# Autodesk Inventor assembly: ASY Beshkino_bio_tank
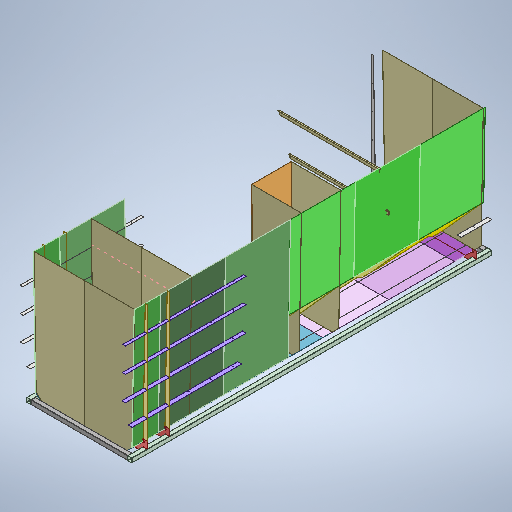
[picture p0: Inventor's stored thumbnail of the model, 512x512]
Saved by Autodesk Inventor 2025 (Build 290162010, 162A)
## iProperties
Created: 2024-07-21
Part Number: ASY Beshkino_bio_tank
Document SubType Name: Assembly
Designer: admin
Mass: 5.81287e+06 g
Surface Area: 2.77755e+06 cm^2
Volume: 3.12018e+06 cm^3
Density: 1.86299 g/cm^3
Author: admin
## Documents named in this file (29)
- C:\Users\user\YandexDisk\домашниий пк\Inventor\BSH_Beshkino_bio_tank\ASY Beshkino_bio_tank.iam
- C:\Users\user\YandexDisk\домашниий пк\Inventor\BSH_Beshkino_bio_tank\BSH 000 dim Beshkino_bio_tank.ipt
- C:\Users\user\YandexDisk\домашниий пк\Inventor\BSH_Beshkino_bio_tank\BSH 010 floor 1.ipt
- C:\Users\user\YandexDisk\домашниий пк\Inventor\BSH_Beshkino_bio_tank\BSH 021 rib 1.ipt
- C:\Users\user\YandexDisk\домашниий пк\Inventor\BSH_Beshkino_bio_tank\BSH 022 rib 2.ipt
- C:\Users\user\YandexDisk\домашниий пк\Inventor\BSH_Beshkino_bio_tank\BSH 061 tube 1.ipt
- C:\Users\user\YandexDisk\домашниий пк\Inventor\BSH_Beshkino_bio_tank\BSH 031 nose 1.ipt
- C:\Users\user\YandexDisk\домашниий пк\Inventor\BSH_Beshkino_bio_tank\BSH 032 board 2.ipt
- C:\Users\user\YandexDisk\домашниий пк\Inventor\BSH_Beshkino_bio_tank\BSH 033 board 3.ipt
- C:\Users\user\YandexDisk\домашниий пк\Inventor\BSH_Beshkino_bio_tank\BSH 041 stringer 1.ipt
- C:\Users\user\YandexDisk\домашниий пк\Inventor\BSH_Beshkino_bio_tank\BSH 039 back 9.ipt
- C:\Users\user\YandexDisk\домашниий пк\Inventor\BSH_Beshkino_bio_tank\BSH 041 stringer floor.ipt
- C:\Users\user\YandexDisk\домашниий пк\Inventor\BSH_Beshkino_bio_tank\BSH 062 tube 2.ipt
- C:\Users\user\YandexDisk\домашниий пк\Inventor\BSH_Beshkino_bio_tank\BSH 042 stringer 2.ipt
- C:\Users\user\YandexDisk\домашниий пк\Inventor\BSH_Beshkino_bio_tank\BSH 043 stringer 3.ipt
- C:\Users\user\YandexDisk\домашниий пк\Inventor\BSH_Beshkino_bio_tank\BSH 044 stringer 4.ipt
- C:\Users\user\YandexDisk\домашниий пк\Inventor\BSH_Beshkino_bio_tank\BSH 020 rib 1.ipt
- C:\Users\user\YandexDisk\домашниий пк\Inventor\BSH_Beshkino_bio_tank\BSH 042 stringer floor.ipt
- C:\Users\user\YandexDisk\домашниий пк\Inventor\BSH_Beshkino_bio_tank\BSH 045 stringer 1.ipt
- C:\Users\user\YandexDisk\домашниий пк\Inventor\BSH_Beshkino_bio_tank\BSH 045 stringer 5.ipt
- C:\Users\user\YandexDisk\домашниий пк\Inventor\BSH_Beshkino_bio_tank\BSH 033 board cone 3.ipt
- C:\Users\user\YandexDisk\домашниий пк\Inventor\BSH_Beshkino_bio_tank\BSH 034 board cone 4.ipt
- C:\Users\user\YandexDisk\домашниий пк\Inventor\BSH_Beshkino_bio_tank\BSH 035 divider 1.ipt
- C:\Users\user\YandexDisk\домашниий пк\Inventor\BSH_Beshkino_bio_tank\BSH 036 divider 2.ipt
- C:\Users\user\YandexDisk\домашниий пк\Inventor\BSH_Beshkino_bio_tank\BSH 012 floor 2.ipt
- C:\Users\user\YandexDisk\домашниий пк\Inventor\BSH_Beshkino_bio_tank\BSH 037 cone 3.ipt
- C:\Users\user\YandexDisk\домашниий пк\Inventor\BSH_Beshkino_bio_tank\BSH 013 floor 3.ipt
- C:\Users\user\YandexDisk\домашниий пк\Inventor\BSH_Beshkino_bio_tank\BSH 015 board cone 5.ipt
- C:\Users\user\YandexDisk\домашниий пк\Inventor\BSH_Beshkino_bio_tank\BSH 038 divider.ipt
## Components (70 placed, 34 different names)
1. BSH 000 dim Beshkino_bio_tank.ipt:1
2. BSH 022 rib 2.ipt:1 — Rigid:3, Mate:8, Rigid:27, Rigid:28, Rigid:29, Rigid:30
3. BSH 061 tube 1.ipt:1 — Mate:1, Rigid:1, Mate:3
4. BSH 061 tube 1.ipt:2 — Mate:2, Rigid:1, Mate:4, Flush:3, Flush:4, Rigid:14, Rigid:15, Mate:20, Mate:21
5. BSH 062 tube 2.ipt:1 — Rigid:14, Mate:19
6. BSH 062 tube 2.ipt:2 — Rigid:15
7. BSH 010 floor 1.ipt:2 — Rigid:4, Rigid:5, Mate:39
8. BSH 010 floor 1.ipt:3 — Rigid:5, Mate:9, Rigid:65, Mate:47, Mate:54
9. BSH 010 floor 1.ipt:1 — Mate:5, Mate:6, Rigid:4, Mate:7, Flush:4, Mate:10, Flush:5, Flush:11
10. BSH 031 nose 1.ipt:1 — Mate:10, Flush:5, Mate:11, Rigid:11
11. BSH 032 board 2.ipt:1 — Mate:8, Mate:9, Rigid:8, Rigid:58
12. BSH 033 board 3.ipt:1 — Rigid:8, Flush:10, Flush:11
13. BSH 031 nose 1.ipt:2 — Rigid:11, Rigid:53
14. BSH 039 back 9.ipt:1 — Rigid:68, Rigid:69
15. BSH 022 rib 2.ipt:2 — Rigid:16, Rigid:31, Rigid:32, Rigid:33, Rigid:34, Mate:38
16. BSH 021 rib 1.ipt:1 — Mate:4, Flush:3, Mate:5, Mate:6, Rigid:3, Rigid:9, Rigid:16, Rigid:20, Rigid:22, Rigid:24, Rigid:26, Mate:19
17. BSH 041 stringer floor.ipt:2 — Rigid:22, Rigid:41
18. BSH 041 stringer floor.ipt:3 — Rigid:24, Rigid:42
19. BSH 041 stringer floor.ipt:4 — Rigid:26, Rigid:43
20. BSH 041 stringer floor.ipt:5 — Rigid:35, Rigid:36
21. BSH 041 stringer floor.ipt:6 — Rigid:36
22. BSH 041 stringer floor:10 — Rigid:41
23. BSH 041 stringer floor:11
24. BSH 041 stringer floor:12 — Rigid:42
25. BSH 041 stringer floor:14 — Rigid:43
26. BSH 041 stringer floor:13
27. BSH 041 stringer floor:15
28. BSH 041 stringer floor.ipt:1 — Rigid:20, Rigid:35
29. BSH 042 stringer floor:1 — Rigid:37
30. BSH 042 stringer floor:2 — Rigid:44
31. BSH 042 stringer floor:3 — Rigid:45
32. BSH 042 stringer floor:4 — Rigid:46
33. BSH 020 rib 1:4 — Mate:20, Mate:21, Rigid:37, Rigid:44, Rigid:45, Rigid:46, Rigid:48
34. BSH 022 rib 2:32 — Rigid:48
35. BSH 045 stringer 1:1
36. BSH 045 stringer 5:1 — Mate:22, Mate:23
37. BSH 031 nose 1:3 — Rigid:55, Mate:22
38. BSH 031 nose 1:4 — Rigid:53
39. BSH 031 nose 1:5 — Rigid:54, Mate:29, Mate:41, Mate:48, Mate:51, Mate:56, Mate:57
40. BSH 031 nose 1:6 — Rigid:54, Rigid:55, Mate:55
41. BSH 033 board cone 3:1 — Mate:26, Rigid:57, Mate:30
42. BSH 031 nose 1:7 — Mate:26, Mate:30
43. BSH 031 nose 1:8 — Flush:8, Mate:40
44. BSH 033 board cone 3:2 — Rigid:57, Mate:29, Mate:41, Mate:46, Angle:1, Mate:49, Mate:50, Mate:52
45. BSH 032 board 2:2 — Rigid:58, Rigid:68
46. BSH 022 rib 2.ipt:3 — Rigid:17
47. BSH 021 rib 1.ipt:2 — Rigid:9, Rigid:17, Rigid:18
48. BSH 022 rib 2.ipt:4 — Rigid:18
49. BSH 044 stringer 4.ipt:1 — Rigid:30
50. BSH 043 stringer 3.ipt:1 — Rigid:29
51. BSH 042 stringer 2.ipt:1 — Rigid:28
52. BSH 041 stringer 1.ipt:1 — Rigid:27
53. BSH 041 stringer 1.ipt:2 — Rigid:31
54. BSH 042 stringer 2.ipt:2 — Rigid:32
55. BSH 043 stringer 3.ipt:2 — Rigid:33
56. BSH 044 stringer 4.ipt:2 — Rigid:34
57. BSH 034 board cone 4:1 — Rigid:62, Mate:43, Mate:51, Mate:52, Mate:53
58. BSH 034 board cone 4:2 — Rigid:62
59. BSH 035 divider 1:1 — Mate:44
60. BSH 036 divider 2:1
61. BSH 012 floor 2:1 — Rigid:65, Rigid:66, Mate:42, Angle:1, Mate:49, Mate:53
62. BSH 037 cone 3:1 — Mate:42, Mate:43, Mate:50
63. BSH 033 board 3:2 — Rigid:64, Flush:10
64. BSH 012 floor 2:2 — Rigid:66, Rigid:67
65. BSH 013 floor 3:1 — Rigid:67, Mate:40
66. BSH 039 back 9:2 — Rigid:69, Rigid:70
67. BSH 039 back 9:3 — Rigid:70
68. BSH 015 board cone 5:1 — Mate:46, Mate:47, Mate:48
69. BSH 038 divider:1 — Mate:54, Mate:55, Mate:56, Mate:57
70. BSH 032 board 2:4 — Mate:38, Mate:39, Rigid:64
## Component patterns: (1 elements, first: BSH 032 board 2:4)
## Relationships (97: WeldJoint 52, Mate 38, Flush 6, Angle 1)
- Mate:1: BSH 061 tube 1.ipt:1
- Mate:2: BSH 061 tube 1.ipt:2
- Rigid:1 [WeldJoint] (-2400 mm): BSH 061 tube 1.ipt:1 ↔ BSH 061 tube 1.ipt:2
- Mate:3: BSH 061 tube 1.ipt:1
- Mate:4: BSH 061 tube 1.ipt:2 ↔ BSH 021 rib 1.ipt:1
- Flush:3: BSH 061 tube 1.ipt:2 ↔ BSH 021 rib 1.ipt:1
- Mate:5: BSH 010 floor 1.ipt:1 ↔ BSH 021 rib 1.ipt:1
- Mate:6: BSH 010 floor 1.ipt:1 ↔ BSH 021 rib 1.ipt:1
- Rigid:3 [WeldJoint]: BSH 022 rib 2.ipt:1 ↔ BSH 021 rib 1.ipt:1
- Rigid:4 [WeldJoint]: BSH 010 floor 1.ipt:2 ↔ BSH 010 floor 1.ipt:1
- Rigid:5 [WeldJoint]: BSH 010 floor 1.ipt:2 ↔ BSH 010 floor 1.ipt:3
- Mate:7: BSH 010 floor 1.ipt:1
- Flush:4 (100 mm): BSH 061 tube 1.ipt:2 ↔ BSH 010 floor 1.ipt:1
- Mate:8: BSH 022 rib 2.ipt:1 ↔ BSH 032 board 2.ipt:1
- Mate:9: BSH 010 floor 1.ipt:3 ↔ BSH 032 board 2.ipt:1
- Rigid:8 [WeldJoint]: BSH 032 board 2.ipt:1 ↔ BSH 033 board 3.ipt:1
- Rigid:9 [WeldJoint] (-500 mm): BSH 021 rib 1.ipt:1 ↔ BSH 021 rib 1.ipt:2
- Mate:10: BSH 010 floor 1.ipt:1 ↔ BSH 031 nose 1.ipt:1
- Flush:5 (10 mm): BSH 010 floor 1.ipt:1 ↔ BSH 031 nose 1.ipt:1
- Mate:11: BSH 031 nose 1.ipt:1
- Rigid:11 [WeldJoint]: BSH 031 nose 1.ipt:1 ↔ BSH 031 nose 1.ipt:2
- Rigid:14 [WeldJoint]: BSH 061 tube 1.ipt:2 ↔ BSH 062 tube 2.ipt:1
- Rigid:15 [WeldJoint]: BSH 061 tube 1.ipt:2 ↔ BSH 062 tube 2.ipt:2
- Rigid:16 [WeldJoint]: BSH 022 rib 2.ipt:2 ↔ BSH 021 rib 1.ipt:1
- Rigid:17 [WeldJoint]: BSH 022 rib 2.ipt:3 ↔ BSH 021 rib 1.ipt:2
- Rigid:18 [WeldJoint]: BSH 021 rib 1.ipt:2 ↔ BSH 022 rib 2.ipt:4
- Rigid:20 [WeldJoint] (2 mm): BSH 021 rib 1.ipt:1 ↔ BSH 041 stringer floor.ipt:1
- Rigid:22 [WeldJoint] (2 mm): BSH 021 rib 1.ipt:1 ↔ BSH 041 stringer floor.ipt:2
- Rigid:24 [WeldJoint]: BSH 021 rib 1.ipt:1 ↔ BSH 041 stringer floor.ipt:3
- Rigid:26 [WeldJoint] (2 mm): BSH 021 rib 1.ipt:1 ↔ BSH 041 stringer floor.ipt:4
- Rigid:27 [WeldJoint] (2 mm): BSH 022 rib 2.ipt:1 ↔ BSH 041 stringer 1.ipt:1
- Rigid:28 [WeldJoint] (2 mm): BSH 022 rib 2.ipt:1 ↔ BSH 042 stringer 2.ipt:1
- Rigid:29 [WeldJoint] (2 mm): BSH 022 rib 2.ipt:1 ↔ BSH 043 stringer 3.ipt:1
- Rigid:30 [WeldJoint] (2 mm): BSH 022 rib 2.ipt:1 ↔ BSH 044 stringer 4.ipt:1
- Rigid:31 [WeldJoint] (2 mm): BSH 022 rib 2.ipt:2 ↔ BSH 041 stringer 1.ipt:2
- Rigid:32 [WeldJoint] (2 mm): BSH 022 rib 2.ipt:2 ↔ BSH 042 stringer 2.ipt:2
- Rigid:33 [WeldJoint] (2 mm): BSH 022 rib 2.ipt:2 ↔ BSH 043 stringer 3.ipt:2
- Rigid:34 [WeldJoint] (2 mm): BSH 022 rib 2.ipt:2 ↔ BSH 044 stringer 4.ipt:2
- Mate:19 (248.5 mm): BSH 062 tube 2.ipt:1 ↔ BSH 021 rib 1.ipt:1
- Rigid:35 [WeldJoint]: BSH 041 stringer floor.ipt:5 ↔ BSH 041 stringer floor.ipt:1
- Rigid:36 [WeldJoint]: BSH 041 stringer floor.ipt:5 ↔ BSH 041 stringer floor.ipt:6
- Mate:20: BSH 061 tube 1.ipt:2 ↔ BSH 020 rib 1:4
- Mate:21: BSH 061 tube 1.ipt:2 ↔ BSH 020 rib 1:4
- Rigid:37 [WeldJoint] (2 mm): BSH 042 stringer floor:1 ↔ BSH 020 rib 1:4
- [WeldJoint]: BSH 041 stringer floor:10 ↔ BSH 041 stringer floor:11
- [WeldJoint]: BSH 041 stringer floor:12 ↔ BSH 041 stringer floor:13
- [WeldJoint]: BSH 041 stringer floor:14 ↔ BSH 041 stringer floor:15
- Rigid:41 [WeldJoint]: BSH 041 stringer floor.ipt:2 ↔ BSH 041 stringer floor:10
- Rigid:42 [WeldJoint]: BSH 041 stringer floor.ipt:3 ↔ BSH 041 stringer floor:12
- Rigid:43 [WeldJoint]: BSH 041 stringer floor.ipt:4 ↔ BSH 041 stringer floor:14
- Rigid:44 [WeldJoint] (2 mm): BSH 042 stringer floor:2 ↔ BSH 020 rib 1:4
- Rigid:45 [WeldJoint] (2 mm): BSH 042 stringer floor:3 ↔ BSH 020 rib 1:4
- Rigid:46 [WeldJoint] (2 mm): BSH 042 stringer floor:4 ↔ BSH 020 rib 1:4
- Rigid:48 [WeldJoint]: BSH 020 rib 1:4 ↔ BSH 022 rib 2:32
- Mate:22: BSH 045 stringer 5:1 ↔ BSH 031 nose 1:3
- Mate:23: BSH 045 stringer 5:1
- [WeldJoint]: BSH 031 nose 1:3 ↔ BSH 031 nose 1:4
- Rigid:53 [WeldJoint] (1300 mm): BSH 031 nose 1.ipt:2 ↔ BSH 031 nose 1:4
- Rigid:54 [WeldJoint] (900 mm): BSH 031 nose 1:5 ↔ BSH 031 nose 1:6
- Rigid:55 [WeldJoint] (2500 mm): BSH 031 nose 1:3 ↔ BSH 031 nose 1:6
- [WeldJoint]: BSH 031 nose 1:7 ↔ BSH 031 nose 1:8
- Flush:8: BSH 031 nose 1:8
- Mate:26: BSH 033 board cone 3:1 ↔ BSH 031 nose 1:7
- Rigid:57 [WeldJoint]: BSH 033 board cone 3:1 ↔ BSH 033 board cone 3:2
- Mate:29: BSH 031 nose 1:5 ↔ BSH 033 board cone 3:2
- Mate:30: BSH 033 board cone 3:1 ↔ BSH 031 nose 1:7
- Rigid:58 [WeldJoint]: BSH 032 board 2.ipt:1 ↔ BSH 032 board 2:2
- Rigid:62 [WeldJoint]: BSH 034 board cone 4:1 ↔ BSH 034 board cone 4:2
- Mate:38: BSH 022 rib 2.ipt:2 ↔ BSH 032 board 2:4
- Mate:39: BSH 010 floor 1.ipt:2 ↔ BSH 032 board 2:4
- Rigid:64 [WeldJoint]: BSH 033 board 3:2 ↔ BSH 032 board 2:4
- Flush:10: BSH 033 board 3.ipt:1 ↔ BSH 033 board 3:2
- Flush:11: BSH 010 floor 1.ipt:1 ↔ BSH 033 board 3.ipt:1
- Rigid:65 [WeldJoint]: BSH 010 floor 1.ipt:3 ↔ BSH 012 floor 2:1
- Rigid:66 [WeldJoint]: BSH 012 floor 2:1 ↔ BSH 012 floor 2:2
- Rigid:67 [WeldJoint]: BSH 012 floor 2:2 ↔ BSH 013 floor 3:1
- Mate:40: BSH 031 nose 1:8 ↔ BSH 013 floor 3:1
- Mate:41: BSH 031 nose 1:5 ↔ BSH 033 board cone 3:2
- Rigid:68 [WeldJoint]: BSH 039 back 9.ipt:1 ↔ BSH 032 board 2:2
- Rigid:69 [WeldJoint]: BSH 039 back 9.ipt:1 ↔ BSH 039 back 9:2
- Rigid:70 [WeldJoint]: BSH 039 back 9:2 ↔ BSH 039 back 9:3
- Mate:42: BSH 012 floor 2:1 ↔ BSH 037 cone 3:1
- Mate:43: BSH 034 board cone 4:1 ↔ BSH 037 cone 3:1
- Mate:44: BSH 035 divider 1:1
- Mate:46: BSH 033 board cone 3:2 ↔ BSH 015 board cone 5:1
- Mate:47: BSH 010 floor 1.ipt:3 ↔ BSH 015 board cone 5:1
- Mate:48: BSH 031 nose 1:5 ↔ BSH 015 board cone 5:1
- Angle:1 (132 deg): BSH 033 board cone 3:2 ↔ BSH 012 floor 2:1
- Mate:49: BSH 033 board cone 3:2 ↔ BSH 012 floor 2:1
- Mate:50: BSH 033 board cone 3:2 ↔ BSH 037 cone 3:1
- Mate:51: BSH 031 nose 1:5 ↔ BSH 034 board cone 4:1
- Mate:52 (100 mm): BSH 033 board cone 3:2 ↔ BSH 034 board cone 4:1
- Mate:53: BSH 034 board cone 4:1 ↔ BSH 012 floor 2:1
- Mate:54: BSH 010 floor 1.ipt:3 ↔ BSH 038 divider:1
- Mate:55: BSH 031 nose 1:6 ↔ BSH 038 divider:1
- Mate:56 (-10 mm): BSH 031 nose 1:5 ↔ BSH 038 divider:1
- Mate:57 (-50 mm): BSH 031 nose 1:5 ↔ BSH 038 divider:1
## Named parameters: d102_d89 = 0 mm, d103_d89 = 0 mm, d104_d89 = 0 mm, d118_d31 = 0 mm, d124_d31 = 0 mm
